# Autodesk Inventor assembly: sled plexi
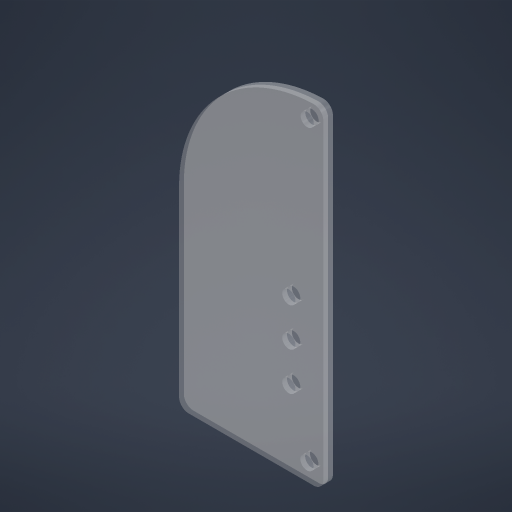
[picture p0: Inventor's stored thumbnail of the model, 512x512]
Saved by Autodesk Inventor 2023 (Build 270158000, 158)
## iProperties
Created: 2023-08-07
Part Number: sled plexi
Document SubType Name: Assembly
Designer: srbel
Author: srbel
## Documents named in this file (2)
- C:\CAD\OverUnderCAD\Drive\sled plexi.iam
- C:\CAD Robotics Season 23-24\sleds.ipt
## Components (2 placed, 1 different names)
1. sleds:1 — Insert:1, Insert:2
2. sleds:2 — Insert:1, Insert:2
## Relationships (2: Insert 2)
- Insert:1: sleds:1 ↔ sleds:2
- Insert:2: sleds:1 ↔ sleds:2
